# Autodesk Inventor assembly: V4.0-trebuchet-printable
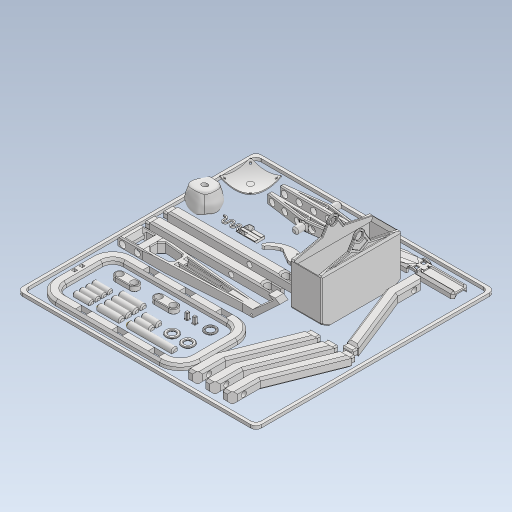
[picture p0: Inventor's stored thumbnail of the model, 512x512]
Saved by Autodesk Inventor 2023 (Build 270158030, 158C)
## iProperties
Created: 2024-12-20
Part Number: V4.0-trebuchet-printable
Document SubType Name: Assembly
Designer: Imogen Heard
Author: Imogen Heard
## Documents named in this file (26)
- C:\Users\dheard\Documents\0004-inventor\3D-CAD-main\trebuchet\V4.0-trebuchet-printable.iam
- C:\Users\dheard\Documents\0004-inventor\3D-CAD-main\trebuchet\pins.ipt
- C:\Users\dheard\Documents\0004-inventor\3D-CAD-main\trebuchet\bolder.ipt
- C:\Users\dheard\Documents\0004-inventor\3D-CAD-main\trebuchet\sling.ipt
- C:\Users\dheard\Documents\0004-inventor\3D-CAD-main\unicorn-horn\washers.ipt
- C:\Users\dheard\Documents\0004-inventor\3D-CAD-main\trebuchet\throw-ring.ipt
- C:\Users\dheard\Documents\0004-inventor\3D-CAD-main\trebuchet\border.ipt
- C:\Users\dheard\Documents\0004-inventor\3D-CAD-main\trebuchet\baseplate.ipt
- C:\Users\dheard\Documents\0004-inventor\3D-CAD-main\trebuchet\V4-upright-A.ipt
- C:\Users\dheard\Documents\0004-inventor\3D-CAD-main\trebuchet\V4-a-frame-A.ipt
- C:\Users\dheard\Documents\0004-inventor\3D-CAD-main\trebuchet\V4-pivot-A.ipt
- C:\Users\dheard\Documents\0004-inventor\3D-CAD-main\trebuchet\V4-throw-arm.ipt
- C:\Users\dheard\Documents\0004-inventor\3D-CAD-main\trebuchet\V4-ratchet.ipt
- C:\Users\dheard\Documents\0004-inventor\3D-CAD-main\trebuchet\V4-counterweight.ipt
- C:\Users\dheard\Documents\0004-inventor\3D-CAD-main\trebuchet\V4-pivot-B.ipt
- C:\Users\dheard\Documents\0004-inventor\3D-CAD-main\trebuchet\V4-upright-B.ipt
- C:\Users\dheard\Documents\0004-inventor\3D-CAD-main\trebuchet\V4-a-frame-B.ipt
- C:\Users\dheard\Documents\0004-inventor\3D-CAD-main\trebuchet\V4-a-frame-C.ipt
- C:\Users\dheard\Documents\0004-inventor\3D-CAD-main\trebuchet\V4-a-frame-D.ipt
- C:\Users\dheard\Documents\0004-inventor\3D-CAD-main\trebuchet\V4-spacer-A.ipt
- C:\Users\dheard\Documents\0004-inventor\3D-CAD-main\trebuchet\V4-spacer-B.ipt
- C:\Users\dheard\Documents\0004-inventor\3D-CAD-main\trebuchet\v4-latch.ipt
- C:\Users\dheard\Documents\0004-inventor\3D-CAD-main\trebuchet\V4-pegs.ipt
- C:\Users\dheard\Documents\0004-inventor\3D-CAD-main\trebuchet\V4-ramp.ipt
- C:\Users\dheard\Documents\0004-inventor\3D-CAD-main\trebuchet\V4-slide.ipt
- C:\Users\dheard\Documents\0004-inventor\3D-CAD-main\trebuchet\V4-pegs-part.ipt
## Components (26 placed, 25 different names)
1. pins:1 — Flush:7, Flush:25, Flush:26, Flush:27, Flush:28, Flush:29, Flush:30, Flush:31, Flush:32, Flush:33, Flush:34, Flush:35, Flush:36, Flush:37, Flush:38, Flush:39
2. bolder:1 — Flush:41
3. sling:1 — Flush:40
4. washers:1 — Flush:19
5. washers:2 — Flush:21
6. throw-ring:1 — Flush:18
7. border:1 — Flush:7, Flush:18, Flush:19, Flush:21, Flush:25, Flush:26, Flush:27, Flush:28, Flush:29, Flush:30, Flush:31, Flush:32, Flush:33, Flush:34, Flush:35, Flush:36, Flush:37, Flush:38, Flush:39, Flush:40, Flush:41, Flush:42, Flush:45, Flush:46, Flush:48, Flush:49, Flush:50, Flush:51, Mate:2, Flush:52, Flush:53, Flush:54, Flush:62, Flush:63, Mate:9, Mate:10, Mate:11, Mate:12, Mate:14, Flush:67, Flush:68
8. V4-baseplate:1 — Flush:42, Flush:61, Mate:7, Mate:8, Mate:11, Mate:12, Mate:16
9. V4-upright-A:1 — Flush:53, Mate:3, Mate:9
10. V4-a-frame-A:1 — Flush:54
11. V4-pivot-A:1 — Flush:46, Flush:47, Mate:1
12. V4-throw-arm:1 — Flush:50, Mate:2
13. V4-ratchet:1 — Flush:49
14. V4-counterweight:1 — Flush:51, Mate:10
15. V4-pivot-B:1 — Flush:47, Mate:1
16. V4-upright-B:1 — Flush:52, Mate:3
17. V4-a-frame-B:1 — Mate:6, Flush:58, Flush:65, Mate:14, Flush:67, Mate:16
18. V4-a-frame-C:1 — Flush:66, Flush:68, Mate:15
19. V4-a-frame-D:1 — Mate:6, Flush:58, Flush:65, Flush:66, Mate:15
20. V4-spacer-A:1 — Flush:62, Flush:64
21. V4-spacer-B:1 — Flush:63, Mate:7, Flush:64
22. v4-latch:1 — Flush:44
23. V4-pegs:1 — Flush:44
24. V4-ramp:1 — Flush:45
25. V4-slide:1 — Flush:48
26. V4-pegs-part:1 — Flush:61, Mate:8
## Relationships (55: Flush 42, Mate 13)
- Flush:7: pins:1 ↔ border:1
- Flush:18: throw-ring:1 ↔ border:1
- Flush:19: washers:1 ↔ border:1
- Flush:21: washers:2 ↔ border:1
- Flush:25: pins:1 ↔ border:1
- Flush:26: pins:1 ↔ border:1
- Flush:27: pins:1 ↔ border:1
- Flush:28: pins:1 ↔ border:1
- Flush:29: pins:1 ↔ border:1
- Flush:30: pins:1 ↔ border:1
- Flush:31: pins:1 ↔ border:1
- Flush:32: pins:1 ↔ border:1
- Flush:33: pins:1 ↔ border:1
- Flush:34: pins:1 ↔ border:1
- Flush:35: pins:1 ↔ border:1
- Flush:36: pins:1 ↔ border:1
- Flush:37: pins:1 ↔ border:1
- Flush:38: pins:1 ↔ border:1
- Flush:39: pins:1 ↔ border:1
- Flush:40: sling:1 ↔ border:1
- Flush:41: bolder:1 ↔ border:1
- Flush:42: border:1 ↔ V4-baseplate:1
- Flush:44: v4-latch:1 ↔ V4-pegs:1
- Flush:45: border:1 ↔ V4-ramp:1
- Flush:46: border:1 ↔ V4-pivot-A:1
- Flush:47: V4-pivot-A:1 ↔ V4-pivot-B:1
- Mate:1 (8 mm): V4-pivot-A:1 ↔ V4-pivot-B:1
- Flush:48: border:1 ↔ V4-slide:1
- Flush:49: border:1 ↔ V4-ratchet:1
- Flush:50: border:1 ↔ V4-throw-arm:1
- Flush:51: border:1 ↔ V4-counterweight:1
- Mate:2 (6 mm): border:1 ↔ V4-throw-arm:1
- Flush:52: border:1 ↔ V4-upright-B:1
- Flush:53: border:1 ↔ V4-upright-A:1
- Mate:3 (7 mm): V4-upright-A:1 ↔ V4-upright-B:1
- Flush:54: border:1 ↔ V4-a-frame-A:1
- Mate:6 (6 mm): V4-a-frame-B:1 ↔ V4-a-frame-D:1
- Flush:58: V4-a-frame-B:1 ↔ V4-a-frame-D:1
- Flush:61: V4-baseplate:1 ↔ V4-pegs-part:1
- Flush:62: border:1 ↔ V4-spacer-A:1
- Flush:63: border:1 ↔ V4-spacer-B:1
- Mate:7 (8 mm): V4-baseplate:1 ↔ V4-spacer-B:1
- Flush:64: V4-spacer-A:1 ↔ V4-spacer-B:1
- Mate:8 (11 mm): V4-baseplate:1 ↔ V4-pegs-part:1
- Mate:9 (6 mm): border:1 ↔ V4-upright-A:1
- Mate:10 (35 mm): border:1 ↔ V4-counterweight:1
- Mate:11 (6 mm): border:1 ↔ V4-baseplate:1
- Mate:12 (5 mm): border:1 ↔ V4-baseplate:1
- Flush:65: V4-a-frame-B:1 ↔ V4-a-frame-D:1
- Mate:14 (6 mm): border:1 ↔ V4-a-frame-B:1
- Flush:66: V4-a-frame-C:1 ↔ V4-a-frame-D:1
- Flush:67: border:1 ↔ V4-a-frame-B:1
- Flush:68: border:1 ↔ V4-a-frame-C:1
- Mate:15 (6 mm): V4-a-frame-C:1 ↔ V4-a-frame-D:1
- Mate:16 (5 mm): V4-baseplate:1 ↔ V4-a-frame-B:1
